# Autodesk Inventor assembly: rd
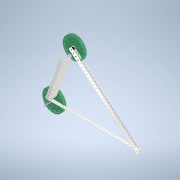
[picture p0: Inventor's stored thumbnail of the model, 180x180]
Saved by Autodesk Inventor 2022.2 (Build 262287000, 287)
## iProperties
Created: 2022-05-26
Part Number: rd
Document SubType Name: Assembly
Designer: Nathan
Author: Nathan
## Documents named in this file (6)
- C:\Users\Natha\Documents\vexcode-projects\TwistedNuts\CAD\rd.iam
- C:\Users\Natha\Documents\Inventor\Content Center Files\R2022\VEX-CAD-Inventor\Structure\C-Channels\Aluminum 1x3x1\Alu C 1x3x1x15.ipt
- C:\Users\Natha\Documents\Inventor\Content Center Files\R2022\VEX-CAD-Inventor\Motion\Gears\HS 84T Gear, Square.ipt
- C:\Users\Natha\Documents\Inventor\Content Center Files\R2022\VEX-CAD-Inventor\Motion\Shaft LS\Shaft LS 3.0 in.ipt
- C:\Users\Natha\Documents\Inventor\Content Center Files\R2022\VEX-CAD-Inventor\Motion\Shaft LS.ipt
- C:\Users\Natha\Documents\Inventor\Content Center Files\R2022\VEX-CAD-Inventor\Structure\C-Channels\Aluminum 1x3x1 Half\Alu Half C 1x3x1x30.ipt
## Components (6 placed, 4 different names)
1. Alu C 1x3x1x15:1 — Mate:1, Mate:2, Mate:3, Mate:4
2. HS 84T Gear, Square:1 — Mate:2, Mate:3, Mate:5, Flush:1, Rotation:1, Mate:6
3. HS 84T Gear, Square:2 — Mate:1, Mate:4, Rotation:1, Mate:7
4. Shaft LS 3.0 in:1 — Mate:5, Flush:1, Angle:1
5. Alu Half C 1x3x1x30:1 — Mate:7, Mate:8
6. Alu Half C 1x3x1x30:2 — Angle:1, Mate:6, Mate:8
## Relationships (11: Mate 8, Flush 1, RelateRotation 1, Angle 1)
- Mate:1: Alu C 1x3x1x15:1 ↔ HS 84T Gear, Square:2
- Mate:2: Alu C 1x3x1x15:1 ↔ HS 84T Gear, Square:1
- Mate:3: Alu C 1x3x1x15:1 ↔ HS 84T Gear, Square:1
- Mate:4: Alu C 1x3x1x15:1 ↔ HS 84T Gear, Square:2
- Mate:5: HS 84T Gear, Square:1 ↔ Shaft LS 3.0 in:1
- Flush:1 (25.4 mm): HS 84T Gear, Square:1 ↔ Shaft LS 3.0 in:1
- Rotation:1 [RelateRotation] (1 ul): HS 84T Gear, Square:1 ↔ HS 84T Gear, Square:2
- Angle:1 (0 deg): Shaft LS 3.0 in:1 ↔ Alu Half C 1x3x1x30:2
- Mate:6: HS 84T Gear, Square:1 ↔ Alu Half C 1x3x1x30:2
- Mate:7: HS 84T Gear, Square:2 ↔ Alu Half C 1x3x1x30:1
- Mate:8: Alu Half C 1x3x1x30:1 ↔ Alu Half C 1x3x1x30:2
